# Autodesk Inventor assembly: TestAssm
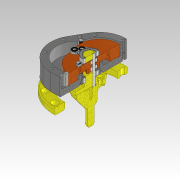
[picture p0: Inventor's stored thumbnail of the model, 180x180]
Saved by Autodesk Inventor 2020 (Build 240168000, 168)
## iProperties
Created: 2021-05-17
Part Number: TestAssm
Document SubType Name: Assembly
Designer: DDeGo
Author: DDeGo
## Documents named in this file (20)
- C:\Users\DDeGo\Documents\Drew\Projects\AirWankelEngine\cad\LiquidPiston V1.7\LiquidPiston_V1_7.iam
- C:\Users\DDeGo\Documents\Drew\Projects\AirWankelEngine\cad\LiquidPiston V1.7\Housing.ipt
- C:\Users\DDeGo\Documents\Drew\Projects\AirWankelEngine\cad\LiquidPiston V1.7\TestAssm\Design Accelerator\Spur Gears1.iam
- C:\Users\DDeGo\Documents\Drew\Projects\AirWankelEngine\cad\LiquidPiston V1.7\Head.ipt
- C:\Users\DDeGo\Documents\Drew\Projects\AirWankelEngine\cad\LiquidPiston V1.7\ApexSeal.ipt
- C:\Users\DDeGo\Documents\Drew\Projects\AirWankelEngine\cad\hardware\2x22 pin.ipt
- C:\Users\DDeGo\Documents\Drew\Projects\AirWankelEngine\cad\LiquidPiston V1.7\FlywheelXL.ipt
- C:\Users\DDeGo\Documents\Drew\Projects\AirWankelEngine\cad\LiquidPiston V1.7\MotorTestBracket.ipt
- C:\Users\DDeGo\Documents\Drew\Projects\AirWankelEngine\cad\LiquidPiston V1.7\2020 Extrusion.ipt
- C:\Users\DDeGo\Documents\Drew\Projects\AirWankelEngine\dyno\Lever.ipt
- C:\Users\DDeGo\Documents\Drew\Projects\AirWankelEngine\dyno\EncoderBracket.ipt
- C:\Users\DDeGo\Documents\Drew\Projects\AirWankelEngine\dyno\Encoder.ipt
- C:\Users\DDeGo\Documents\Drew\Projects\AirWankelEngine\cad\LiquidPiston V1.7\Rotor_NEW.ipt
- C:\Users\DDeGo\Documents\Drew\Projects\AirWankelEngine\cad\LiquidPiston V1.7\TestAssm\Design Accelerator\Spur Gears2.iam
- C:\Users\DDeGo\Documents\Drew\Projects\AirWankelEngine\cad\LiquidPiston V1.7\CamShaft.ipt
- C:\Users\DDeGo\Documents\Drew\Projects\AirWankelEngine\cad\hardware\MR52 Bearing.ipt
- C:\Users\DDeGo\Documents\Drew\Projects\AirWankelEngine\cad\hardware\MR128 bearing.ipt
- C:\Users\DDeGo\Documents\Drew\Projects\AirWankelEngine\cad\LiquidPiston V1.7\Flywheel.ipt
- C:\Users\DDeGo\Documents\Drew\Projects\AirWankelEngine\cad\hardware\oring_4x2x1.ipt
- C:\Users\DDeGo\Documents\Drew\Projects\AirWankelEngine\cad\LiquidPiston V1.7\ValveThing.ipt
## Components (30 placed, 18 different names)
1. Housing:1 — Mate:11, Mate:14, Mate:66, Mate:67, Mate:68, Mate:69, Mate:80, Mate:105, Mate:109, Mate:113, Mate:114, Mate:127
2. Spur Gears:1 [sub-assembly]
3. ApexSeal:1 — Mate:11, Mate:67
4. ApexSeal:2 — Mate:14, Mate:68
5. ApexSeal:3 — Mate:66
6. 2x22 pin:1 — Mate:118, Mate:119, Mate:120, Mate:123
7. Head:1 — Mate:69, Mate:113, Mate:114, Mate:115, Mate:128, Mate:129, Mate:130, Mate:131, Mate:132, Mate:133, Tangent:1, Tangent:2, Tangent:3, Tangent:4, Tangent:5, Tangent:6, Mate:134, Mate:135, Mate:136, Mate:137, Mate:138, Mate:139
8. MotorTestBracket:1 — Mate:80, Mate:82, Flush:8, Flush:9
9. 2020 Extrusion:1 — Mate:82, Flush:8, Flush:9, Mate:89, Flush:10
10. Lever:1
11. EncoderBracket:1 — Mate:89, Flush:10, Mate:90, Mate:91, Mate:92
12. Encoder:1 — Mate:90, Mate:91, Mate:92
13. Rotor_NEW:1 — Mate:105, Mate:106, Mate:107, Flush:12, Flush:13, Rotation:1, Mate:140
14. Spur Gears:2 [sub-assembly]
15. FlywheelXL:2 — Mate:124, Mate:125, Mate:126
16. CamShaft:1 — Flush:14, Mate:117, Mate:118, Mate:123, Rotation:1
17. MR52 Bearing:1 — Mate:106, Flush:12
18. MR128 bearing:1 — Mate:109, Mate:121, Mate:122, Mate:127
19. MR52 Bearing:2 — Mate:107, Flush:13, Mate:119
20. MR128 bearing:2 — Mate:115, Flush:14, Mate:117
21. Flywheel:1 — Mate:120, Mate:121, Mate:122, Mate:124, Mate:125, Mate:126
22. oring_4x2x1:1 — Mate:128, Tangent:6
23. oring_4x2x1:2 — Mate:129, Tangent:4
24. oring_4x2x1:3 — Mate:133, Tangent:5
25. oring_4x2x1:4 — Mate:132, Tangent:3
26. oring_4x2x1:5 — Mate:130, Tangent:1
27. oring_4x2x1:6 — Mate:131, Tangent:2
28. ValveThing:1 — Mate:134, Mate:137, Flush:16
29. ValveThing:2 — Mate:136, Mate:138, Flush:15, Flush:16, Mate:140
30. ValveThing:3 — Mate:135, Mate:139, Flush:15
## Relationships (58: Mate 43, Flush 8, Tangent 6, RelateRotation 1)
- Mate:11 (0.1 mm): Housing:1 ↔ ApexSeal:1
- Mate:14 (0.1 mm): Housing:1 ↔ ApexSeal:2
- Mate:66: Housing:1 ↔ ApexSeal:3
- Mate:67: Housing:1 ↔ ApexSeal:1
- Mate:68: Housing:1 ↔ ApexSeal:2
- Mate:69: Housing:1 ↔ Head:1
- Mate:80: Housing:1 ↔ MotorTestBracket:1
- Mate:82: MotorTestBracket:1 ↔ 2020 Extrusion:1
- Flush:8: MotorTestBracket:1 ↔ 2020 Extrusion:1
- Flush:9 (5 mm): MotorTestBracket:1 ↔ 2020 Extrusion:1
- Mate:89: 2020 Extrusion:1 ↔ EncoderBracket:1
- Flush:10: 2020 Extrusion:1 ↔ EncoderBracket:1
- Mate:90: EncoderBracket:1 ↔ Encoder:1
- Mate:91: EncoderBracket:1 ↔ Encoder:1
- Mate:92: EncoderBracket:1 ↔ Encoder:1
- Mate:105: Housing:1 ↔ Rotor_NEW:1
- Mate:106: Rotor_NEW:1 ↔ MR52 Bearing:1
- Mate:107: Rotor_NEW:1 ↔ MR52 Bearing:2
- Mate:109: Housing:1 ↔ MR128 bearing:1
- Flush:12 (-0.5 mm): Rotor_NEW:1 ↔ MR52 Bearing:1
- Flush:13 (-0.5 mm): Rotor_NEW:1 ↔ MR52 Bearing:2
- Mate:113: Housing:1 ↔ Head:1
- Mate:114: Housing:1 ↔ Head:1
- Mate:115: Head:1 ↔ MR128 bearing:2
- Flush:14: CamShaft:1 ↔ MR128 bearing:2
- Mate:117: CamShaft:1 ↔ MR128 bearing:2
- Mate:118: 2x22 pin:1 ↔ CamShaft:1
- Mate:119: 2x22 pin:1 ↔ MR52 Bearing:2
- Mate:120: 2x22 pin:1 ↔ Flywheel:1
- Mate:121: MR128 bearing:1 ↔ Flywheel:1
- Mate:122: MR128 bearing:1 ↔ Flywheel:1
- Mate:123: 2x22 pin:1 ↔ CamShaft:1
- Rotation:1 [RelateRotation] (0.5 ul): Rotor_NEW:1 ↔ CamShaft:1
- Mate:124: FlywheelXL:2 ↔ Flywheel:1
- Mate:125: FlywheelXL:2 ↔ Flywheel:1
- Mate:126: FlywheelXL:2 ↔ Flywheel:1
- Mate:127: Housing:1 ↔ MR128 bearing:1
- Mate:128: Head:1 ↔ oring_4x2x1:1
- Mate:129: Head:1 ↔ oring_4x2x1:2
- Mate:130: Head:1 ↔ oring_4x2x1:5
- Mate:131: Head:1 ↔ oring_4x2x1:6
- Mate:132: Head:1 ↔ oring_4x2x1:4
- Mate:133: Head:1 ↔ oring_4x2x1:3
- Tangent:1: Head:1 ↔ oring_4x2x1:5
- Tangent:2: Head:1 ↔ oring_4x2x1:6
- Tangent:3: Head:1 ↔ oring_4x2x1:4
- Tangent:4: Head:1 ↔ oring_4x2x1:2
- Tangent:5: Head:1 ↔ oring_4x2x1:3
- Tangent:6: Head:1 ↔ oring_4x2x1:1
- Mate:134: Head:1 ↔ ValveThing:1
- Mate:135: Head:1 ↔ ValveThing:3
- Mate:136: Head:1 ↔ ValveThing:2
- Mate:137: Head:1 ↔ ValveThing:1
- Mate:138: Head:1 ↔ ValveThing:2
- Mate:139: Head:1 ↔ ValveThing:3
- Flush:15: ValveThing:2 ↔ ValveThing:3
- Flush:16: ValveThing:1 ↔ ValveThing:2
- Mate:140: Rotor_NEW:1 ↔ ValveThing:2
